# Autodesk Inventor assembly: !odom_pod
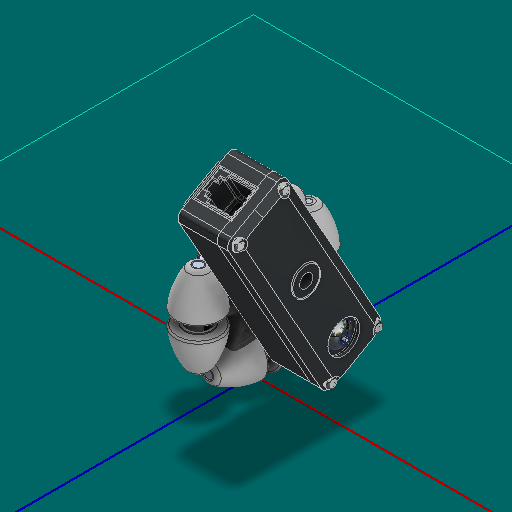
[picture p0: Inventor's stored thumbnail of the model, 512x512]
Saved by Autodesk Inventor 2025 (Build 290162000, 162)
## iProperties
Created: 2024-08-18
Part Number: !odom_pod
Document SubType Name: Assembly
Designer: averey
Author: averey
## Documents named in this file (9)
- C:\Users\avere\vex_robotics_high_stakes\hardware\cad\ATLAS\chassis\odom_pod\!odom_pod.iam
- C:\Users\avere\vex_robotics_high_stakes\hardware\cad\VEX-CAD-Inventor\Motion\Wheels\Omni Wheel\2.00 Omni AS, No Insert.ipt
- C:\Users\avere\vex_robotics_high_stakes\hardware\cad\VEX-CAD-Inventor\Electronics\Sensors\V5 Rotation Sensor.ipt
- C:\Users\avere\vex_robotics_high_stakes\hardware\cad\VEX-CAD-Inventor\Motion\Shaft HS\HS Spacer.ipt
- C:\Users\avere\vex_robotics_high_stakes\hardware\cad\VEX-CAD-Inventor\Motion\HS Shaft Adapter Circle.ipt
- C:\Users\avere\vex_robotics_high_stakes\hardware\cad\VEX-CAD-Inventor\Motion\Shaft HS\HS Spacer\HSpacer .0625.ipt
- C:\Users\avere\vex_robotics_high_stakes\hardware\cad\VEX-CAD-Inventor\Structure\Hardware\Screw Steel - Star\SScrew Star Smooth 1.750.ipt
- C:\Users\avere\vex_robotics_high_stakes\hardware\cad\VEX-CAD-Inventor\Structure\Hardware\Screw Steel - Star.ipt
- C:\Users\avere\vex_robotics_high_stakes\hardware\cad\VEX-CAD-Inventor\Structure\Hardware\Nut Thin Nylock.ipt
## Components (10 placed, 6 different names)
1. 2.00 Omni AS, No Insert:1 — Angle:1, Insert:12, Mate:2, Mate:3, Insert:15
2. V5 Rotation Sensor:1 — Angle:1, Insert:11, Mate:1
3. HSpacer .0625:1 — Insert:12
4. SScrew Star Smooth 1.750:1 — Insert:14
5. HS Shaft Adapter Circle:3 — Insert:11, Mate:1, Insert:14
6. HS Shaft Adapter Circle:4 — Insert:13, Flush:3
7. HS Shaft Adapter Circle:5 — Insert:13, Flush:3, Mate:2, Mate:3, Angle:2, Angle:3
8. HSpacer .0625:2 — Insert:15, Angle:2, Insert:16
9. HSpacer .0625:3 — Insert:16, Angle:3, Insert:17
10. Nut Thin Nylock:1 — Insert:17
## Relationships (16: Insert 8, Angle 3, Mate 3, Flush 2)
- Angle:1 (0 deg): 2.00 Omni AS, No Insert:1 ↔ V5 Rotation Sensor:1
- [Insert]: HS Shaft Adapter Circle:3 ↔ HS Shaft Adapter Circle:4
- [Flush]: HS Shaft Adapter Circle:3 ↔ HS Shaft Adapter Circle:4
- Insert:11: V5 Rotation Sensor:1 ↔ HS Shaft Adapter Circle:3
- Mate:1: V5 Rotation Sensor:1 ↔ HS Shaft Adapter Circle:3
- Insert:12: 2.00 Omni AS, No Insert:1 ↔ HSpacer .0625:1
- Insert:13: HS Shaft Adapter Circle:4 ↔ HS Shaft Adapter Circle:5
- Flush:3: HS Shaft Adapter Circle:4 ↔ HS Shaft Adapter Circle:5
- Mate:2: 2.00 Omni AS, No Insert:1 ↔ HS Shaft Adapter Circle:5
- Mate:3: 2.00 Omni AS, No Insert:1 ↔ HS Shaft Adapter Circle:5
- Insert:14: SScrew Star Smooth 1.750:1 ↔ HS Shaft Adapter Circle:3
- Insert:15: 2.00 Omni AS, No Insert:1 ↔ HSpacer .0625:2
- Angle:2 (0 deg): HS Shaft Adapter Circle:5 ↔ HSpacer .0625:2
- Insert:16: HSpacer .0625:2 ↔ HSpacer .0625:3
- Angle:3 (0 deg): HS Shaft Adapter Circle:5 ↔ HSpacer .0625:3
- Insert:17: HSpacer .0625:3 ↔ Nut Thin Nylock:1
## Named parameters: d21_d14 = 0 mm, d22_d15 = 0 mm
